# Autodesk Inventor assembly: 5x3holder_assembly
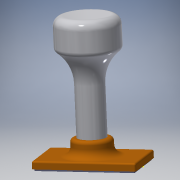
[picture p0: Inventor's stored thumbnail of the model, 180x180]
Saved by Autodesk Inventor 2019 (Build 230136000, 136)
## iProperties
Created: 2019-02-19
Part Number: 5x3holder_assembly
Document SubType Name: Assembly
Designer: jmc
Author: jmc
## Documents named in this file (4)
- C:\Users\l0086\Desktop\Models\Stamp\5x3holder_assembly.iam
- C:\Users\l0086\Desktop\Models\Stamp\holder_nut_5x3.ipt
- C:\Users\l0086\Desktop\Models\Stamp\holder.ipt
- C:\Users\l0086\Desktop\Models\Stamp\stamp5x3.ipt
## Components (3 placed, 3 different names)
1. holder_nut_5x3:1 — Cylindrical:1, Rigid:1
2. holder:1 — Cylindrical:1
3. stamp5x3:1 — Rigid:1
## Relationships (2: CylindricalJoint 1, WeldJoint 1)
- Cylindrical:1: holder_nut_5x3:1 ↔ holder:1
- Rigid:1 [WeldJoint]: holder_nut_5x3:1 ↔ stamp5x3:1
